# Autodesk Inventor assembly: trans-asm-interior
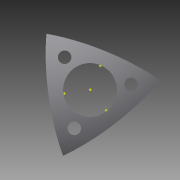
[picture p0: Inventor's stored thumbnail of the model, 180x180]
Saved by Autodesk Inventor 2015 SP2 (Build 190223200, 223)
## iProperties
Created: 2015-05-05
Part Number: trans-asm-interior
Document SubType Name: Assembly
Designer: foote
Mass: 466.005 g
Surface Area: 1246.44 cm^2
Volume: 466.005 cm^3
Density: 1 g/cm^3
Author: foote
## Documents named in this file (2)
- C:\foote\projects\AIR\ommalamp\assembly-2\sect_bottom\trans-asm-bottom.iam
- C:\foote\projects\AIR\ommalamp\assembly-2\sect_bottom\ommatid.ipt
## Components (1 placed, 1 different names)
1. ommatid:1 — Mate:14, Mate:15
## Relationships (2: Mate 2)
- Mate:14: ommatid:1
- Mate:15: ommatid:1
## Named parameters: nut_width = 1.8034 mm, vent_diam = 6.35 mm, vent_inset = 2.54 mm
